# Autodesk Inventor assembly: Cover Assembly Vibrometer
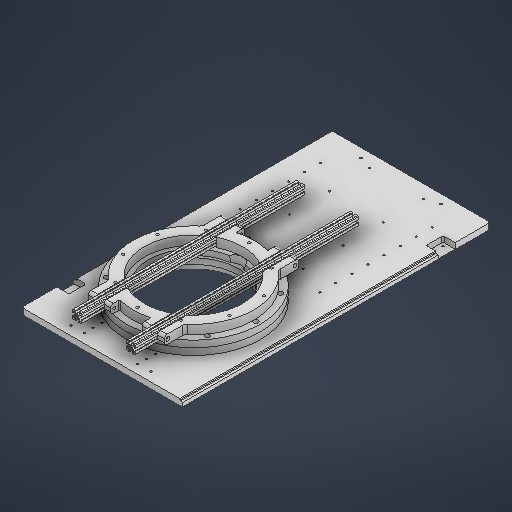
[picture p0: Inventor's stored thumbnail of the model, 512x512]
Saved by Autodesk Inventor 2025 (Build 290162000, 162)
## iProperties
Created: 2025-03-28
Part Number: Cover Assembly Vibrometer
Document SubType Name: Assembly
Designer: mayhe
Author: mayhe
## Documents named in this file (7)
- C:\Users\mayhe\OneDrive\Documents\GitHub\In-situ-monitoring-of-powder-bed-fusion-additive-manufacturing\system_development\Orichalcum\v0.2\Hardware_design\custom-cover\Cover Assembly Vibrometer.iam
- C:\Users\mayhe\OneDrive\Documents\GitHub\In-situ-monitoring-of-powder-bed-fusion-additive-manufacturing\system_development\Orichalcum\v0.2\Hardware_design\custom-cover\cover\Updated Cover (Vibrometer).ipt
- C:\Users\mayhe\OneDrive\Documents\GitHub\In-situ-monitoring-of-powder-bed-fusion-additive-manufacturing\system_development\Mithril\v0.2\Model\300mm Housing 1.ipt
- C:\Users\mayhe\OneDrive\Documents\GitHub\In-situ-monitoring-of-powder-bed-fusion-additive-manufacturing\system_development\Mithril\v0.2\Model\300mm housing 2 Camera.ipt
- C:\Users\mayhe\OneDrive\Documents\GitHub\In-situ-monitoring-of-powder-bed-fusion-additive-manufacturing\system_development\Orichalcum\v0.2\Hardware_design\custom-cover\cylinder-parts\Cylinder 80-20 Spacer_2.ipt
- C:\Users\mayhe\OneDrive\Documents\GitHub\In-situ-monitoring-of-powder-bed-fusion-additive-manufacturing\system_development\Orichalcum\v0.2\Hardware_design\custom-cover\cylinder-parts\Cylinder 80-20 Spacer_1.ipt
- C:\Users\mayhe\OneDrive\Documents\GitHub\In-situ-monitoring-of-powder-bed-fusion-additive-manufacturing\system_development\Orichalcum\v0.2\Hardware_design\custom-cover\8020-parts\20-2020-500-CL.ipt
## Components (9 placed, 6 different names)
1. Updated Cover (Vibrometer):1 — Rotational:1
2. 300mm Housing 1:1 — Rotational:1, Rotational:2
3. 300mm housing 2 Camera:1 — Rotational:2, Rotational:3, Rotational:4, Rotational:5, Rotational:6, Mate:1, Mate:3
4. Cylinder 80-20 Spacer_2:1 — Rotational:3, Flush:2
5. Cylinder 80-20 Spacer_2:2 — Rotational:4, Flush:1, Mate:2
6. Cylinder 80-20 Spacer_1:1 — Rotational:5
7. Cylinder 80-20 Spacer_1:2 — Rotational:6, Mate:4
8. 20-2020-500-CL:1 — Flush:2, Mate:3, Mate:4
9. 20-2020-500-CL:2 — Flush:1, Mate:1, Mate:2
## Relationships (12: RevoluteJoint 6, Mate 4, Flush 2)
- Rotational:1 [RevoluteJoint]: Updated Cover (Vibrometer):1 ↔ 300mm Housing 1:1
- Rotational:2 [RevoluteJoint]: 300mm Housing 1:1 ↔ 300mm housing 2 Camera:1
- Rotational:3 [RevoluteJoint]: 300mm housing 2 Camera:1 ↔ Cylinder 80-20 Spacer_2:1
- Rotational:4 [RevoluteJoint]: 300mm housing 2 Camera:1 ↔ Cylinder 80-20 Spacer_2:2
- Rotational:5 [RevoluteJoint]: 300mm housing 2 Camera:1 ↔ Cylinder 80-20 Spacer_1:1
- Rotational:6 [RevoluteJoint]: 300mm housing 2 Camera:1 ↔ Cylinder 80-20 Spacer_1:2
- Flush:1 (-50 mm): Cylinder 80-20 Spacer_2:2 ↔ 20-2020-500-CL:2
- Mate:1: 300mm housing 2 Camera:1 ↔ 20-2020-500-CL:2
- Mate:2: Cylinder 80-20 Spacer_2:2 ↔ 20-2020-500-CL:2
- Flush:2 (-50 mm): Cylinder 80-20 Spacer_2:1 ↔ 20-2020-500-CL:1
- Mate:3: 300mm housing 2 Camera:1 ↔ 20-2020-500-CL:1
- Mate:4: Cylinder 80-20 Spacer_1:2 ↔ 20-2020-500-CL:1
